# Autodesk Inventor assembly: Cannulation_Asm
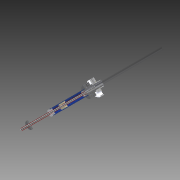
[picture p0: Inventor's stored thumbnail of the model, 180x180]
Saved by Autodesk Inventor 2011 SP2 (Build 150309200, 309)
## iProperties
Created: 2013-09-16
Part Number: Cannulation_Asm
Document SubType Name: Assembly
Designer: sungwook
Author: sungwook
## Documents named in this file (13)
- C:\Users\sungwook\Documents\Inventor\Micron22_top_adj_02082013\Cannulation\Cannulation_Asm.iam
- C:\Users\sungwook\Documents\Inventor\Micron22_top_adj_02082013\Cannulation\tubing_9G.ipt
- C:\Users\sungwook\Documents\Inventor\Micron22_top_adj_02082013\Cannulation\inner_block.ipt
- C:\Users\sungwook\Documents\Inventor\Micron22_top_adj_02082013\Cannulation\tubing_17G.ipt
- C:\Users\sungwook\Documents\Inventor\Micron22_top_adj_02082013\Cannulation\upper_cap.ipt
- C:\Users\sungwook\Documents\Inventor\Micron22_top_adj_02082013\Cannulation\pipette.ipt
- C:\Users\sungwook\Documents\Inventor\Micron22_top_adj_02082013\Cannulation\bottom_cap.ipt
- C:\Users\sungwook\Documents\Inventor\Micron22_top_adj_02082013\Cannulation\Connector.ipt
- C:\Users\sungwook\Documents\Inventor\Micron22_top_adj_02082013\Cannulation\Tool Mount_Rev.ipt
- C:\Users\sungwook\Documents\Inventor\Micron22_top_adj_02082013\Cannulation\tygon_tube.ipt
- C:\Users\sungwook\Documents\Inventor\Micron22_top_adj_02082013\Cannulation\front_block.ipt
- C:\Users\sungwook\Documents\Inventor\Micron22_top_adj_02082013\Cannulation\spring.ipt
- C:\Users\sungwook\Documents\Inventor\Micron22_top_adj_02082013\Cannulation\spring2.ipt
## Components (12 placed, 12 different names)
1. tubing_9G:1 — Mate:1, Mate:2, Mate:4, Mate:7, Mate:8
2. inner_block:1 — Mate:3, Flush:7, Mate:24, Mate:26
3. tubing_17G:1 — Mate:3, Mate:4, Mate:6, Mate:16, Flush:5, Mate:18, Flush:7
4. upper_cap:1 — Mate:1, Mate:2, Mate:24
5. pipette:1 — Mate:6, Mate:14, Mate:15, Mate:17, Mate:21, Eye Dist
6. bottom_cap:1 — Mate:7, Mate:8, Mate:10, Angle:1, Mate:22, Mate:23, Mate:26
7. Connector:1 — Mate:10, Mate:12, Mate:13, Mate:23, Flush:8
8. Tool Mount_Rev:1 — Mate:12, Mate:13, Angle:1
9. tygon_tube:1 — Mate:14, Mate:15, Flush:8
10. front_block:1 — Mate:16, Flush:5, Mate:17, Eye Dist
11. spring:1 — Mate:18
12. spring2:1 — Mate:21, Mate:22
## Relationships (25: Mate 20, Flush 4, Angle 1)
- Mate:1: tubing_9G:1 ↔ upper_cap:1
- Mate:2: tubing_9G:1 ↔ upper_cap:1
- Mate:3: inner_block:1 ↔ tubing_17G:1
- Mate:4: tubing_9G:1 ↔ tubing_17G:1
- Mate:6: tubing_17G:1 ↔ pipette:1
- Mate:7: tubing_9G:1 ↔ bottom_cap:1
- Mate:8: tubing_9G:1 ↔ bottom_cap:1
- Mate:10: bottom_cap:1 ↔ Connector:1
- Mate:12: Connector:1 ↔ Tool Mount_Rev:1
- Mate:13: Connector:1 ↔ Tool Mount_Rev:1
- Mate:14: pipette:1 ↔ tygon_tube:1
- Mate:15 (-5 mm): pipette:1 ↔ tygon_tube:1
- Mate:16: tubing_17G:1 ↔ front_block:1
- Flush:5 (-5.08 mm): tubing_17G:1 ↔ front_block:1
- Mate:17 (20 mm): pipette:1 ↔ front_block:1
- Angle:1 (0 deg): bottom_cap:1 ↔ Tool Mount_Rev:1
- Mate:18: tubing_17G:1 ↔ spring:1
- Mate:21: pipette:1 ↔ spring2:1
- Mate:22: bottom_cap:1 ↔ spring2:1
- Flush:7 (13.0302 mm): inner_block:1 ↔ tubing_17G:1
- Mate:23: bottom_cap:1 ↔ Connector:1
- Flush:8: Connector:1 ↔ tygon_tube:1
- Mate:24: inner_block:1 ↔ upper_cap:1
- Mate:26 (3.429 mm): inner_block:1 ↔ bottom_cap:1
- Eye Dist [Flush] (-8 mm): pipette:1 ↔ front_block:1
